# Autodesk Inventor assembly: 조립
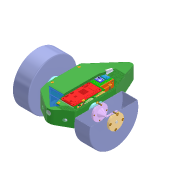
[picture p0: Inventor's stored thumbnail of the model, 180x180]
Saved by Autodesk Inventor 2020 (Build 240168000, 168)
## iProperties
Created: 2020-05-28
Part Number: 조립
Document SubType Name: Assembly
Designer: Miji
Author: Miji
## Documents named in this file (25)
- C:\Users\82102\OneDrive\바탕 화면\개인자료\졸업과제\설계\로봇\모델링 1.2\조립.iam
- C:\Users\82102\OneDrive\바탕 화면\개인자료\졸업과제\설계\로봇\모델링 1.2\본체 조립.iam
- C:\Users\82102\OneDrive\바탕 화면\개인자료\졸업과제\설계\로봇\모델링 1.2\바퀴 서브 조립.iam
- C:\Users\82102\OneDrive\바탕 화면\개인자료\졸업과제\설계\로봇\모델링 1.2\볼.ipt
- C:\Users\82102\OneDrive\바탕 화면\개인자료\졸업과제\설계\로봇\모델링 1.2\전자부품\모터.ipt
- C:\Users\82102\OneDrive\바탕 화면\개인자료\졸업과제\설계\로봇\모델링 1.2\전자부품\건전지.ipt
- C:\Users\82102\OneDrive\바탕 화면\개인자료\졸업과제\설계\로봇\모델링 1.2\전자부품\충방전\충방전.iam
- C:\Users\82102\OneDrive\바탕 화면\개인자료\졸업과제\설계\로봇\모델링 1.2\전자부품\모터드라이버\Motor Driver.ipt
- C:\Users\82102\OneDrive\바탕 화면\개인자료\졸업과제\설계\로봇\모델링 1.2\지름 핸들러.ipt
- C:\Users\82102\OneDrive\바탕 화면\개인자료\졸업과제\설계\로봇\모델링 1.2\바퀴 스퍼기어.ipt
- C:\Users\82102\OneDrive\바탕 화면\개인자료\졸업과제\설계\로봇\모델링 1.2\led 창.ipt
- C:\Users\82102\OneDrive\바탕 화면\개인자료\졸업과제\설계\로봇\모델링 1.2\카메라 창.ipt
- C:\Users\82102\OneDrive\바탕 화면\개인자료\졸업과제\설계\로봇\모델링 1.2\전자부품\카메라.ipt
- C:\Users\82102\OneDrive\바탕 화면\개인자료\졸업과제\설계\로봇\모델링 1.2\전자부품\led.ipt
- C:\Users\82102\OneDrive\바탕 화면\개인자료\졸업과제\설계\로봇\모델링 1.2\전자부품\자이로센서\MPU-9255.iam
- C:\Users\82102\OneDrive\바탕 화면\개인자료\졸업과제\설계\로봇\모델링 1.2\전자부품\아두이노 프로미니\Pro-Mini.ipt
- C:\Users\82102\OneDrive\바탕 화면\개인자료\졸업과제\설계\로봇\모델링 1.2\전자부품\로직 ic\IC CD4017.ipt
- C:\Users\82102\OneDrive\바탕 화면\개인자료\졸업과제\설계\로봇\모델링 1.2\전자부품\고도 센서\bmp180.ipt
- C:\Users\82102\OneDrive\바탕 화면\개인자료\졸업과제\설계\로봇\모델링 1.2\전자부품\raspberry-pi-zero-w\RaspberryPiZeroW.ipt
- C:\Users\82102\OneDrive\바탕 화면\개인자료\졸업과제\설계\로봇\모델링 1.2\전자부품\gps\ublox NEO-6M.iam
- C:\Users\82102\OneDrive\바탕 화면\개인자료\졸업과제\설계\로봇\모델링 1.2\전자부품\브레드 보드\20x53.ipt
- C:\Users\82102\OneDrive\바탕 화면\개인자료\졸업과제\설계\로봇\모델링 1.2\전자부품\브레드 보드\55x60.ipt
- C:\Users\82102\OneDrive\바탕 화면\개인자료\졸업과제\설계\로봇\모델링 1.2\본체 글라스.ipt
- C:\Users\82102\OneDrive\바탕 화면\개인자료\졸업과제\설계\로봇\모델링 1.2\전자부품\5v 승압 회로\Step Up.ipt
- C:\Users\82102\OneDrive\바탕 화면\개인자료\졸업과제\설계\로봇\모델링 1.2\전자부품\gps\Antenna.ipt
## Components (31 placed, 24 different names)
1. 본체 조립:1 [sub-assembly] — 메이트:1, 메이트:2, 메이트:3, 메이트:4, 메이트:5, 메이트:6, 메이트:7, 메이트:8, 메이트:9, 메이트:10, 메이트:11, 메이트:12, 메이트:13, 메이트:14, 메이트:15, 메이트:16, 메이트:17, 메이트:18, 메이트:19, 메이트:23, 메이트:24, 메이트:25, 플러쉬:1, 메이트:30, 메이트:31, 메이트:32, 메이트:33, 접선:1, 메이트:34, 각도:1, 메이트:35, 메이트:36, 플러쉬:4, 메이트:37, 메이트:38, 각도:2, 각도:3, 메이트:39, 메이트:40, 메이트:41, 메이트:42, 각도:4, 메이트:43, 각도:5, 플러쉬:5, 메이트:50, 메이트:51, 메이트:52, 각도:8, 각도:9, 메이트:58, 메이트:59, 메이트:60, 메이트:61, 메이트:62, 플러쉬:6
2. 바퀴 서브 조립:1 [sub-assembly] — 메이트:1, 메이트:2, 플러쉬:3, 회전:1
3. 바퀴 서브 조립:2 [sub-assembly] — 메이트:3, 메이트:4, 플러쉬:2, 회전:2
4. 바퀴 스퍼기어:2 — 메이트:29, 플러쉬:2, 회전:2
5. 바퀴 스퍼기어:1 — 메이트:28, 플러쉬:3, 회전:1
6. 지름 핸들러:1 — 메이트:21, 메이트:22
7. Antenna:1 — 메이트:61, 메이트:62, 플러쉬:6
8. 20x53:1 — 메이트:39, 메이트:40, 메이트:41, 메이트:53, 메이트:54, 메이트:56, 메이트:57
9. 55x60:1 — 메이트:42, 각도:4, 메이트:43, 메이트:44, 메이트:45, 메이트:46, 각도:6, 메이트:47, 메이트:48, 메이트:49, 각도:7
10. Step Up:1 — 메이트:50, 메이트:51, 메이트:52
11. MPU-9255:1 [sub-assembly] — 메이트:53, 메이트:54, 각도:8
12. Pro-Mini:1 — 메이트:46, 각도:6, 메이트:47
13. IC CD4017:1 — 메이트:48, 메이트:49, 각도:7
14. bmp180:2 — 메이트:56, 메이트:57, 각도:9
15. RaspberryPiZeroW:1 — 메이트:44, 각도:5, 메이트:45
16. ublox NEO-6M:1 [sub-assembly] — 메이트:58, 메이트:59, 메이트:60
17. led:1 — 메이트:36, 플러쉬:4, 각도:3
18. led:2 — 메이트:37, 메이트:38, 각도:2
19. 카메라:1 — 메이트:34, 각도:1, 메이트:35
20. 모터:1 — 메이트:9, 메이트:10, 메이트:11, 메이트:29
21. 모터:2 — 메이트:12, 메이트:13, 메이트:14, 메이트:21, 메이트:22
22. 모터:3 — 메이트:6, 메이트:7, 메이트:8, 메이트:28
23. 건전지:1 — 메이트:15, 메이트:16
24. 충방전:1 [sub-assembly] — 메이트:17, 메이트:18, 메이트:19
25. Motor Driver:1 — 메이트:25, 메이트:26, 메이트:27, 플러쉬:1
26. Motor Driver:2 — 메이트:23, 메이트:24, 메이트:26, 메이트:27
27. 볼:1 — 메이트:5
28. 본체 글라스:1 — 플러쉬:5
29. led 창:1 — 메이트:30
30. led 창:2 — 메이트:31, 메이트:32
31. 카메라 창:1 — 메이트:33, 접선:1
## Relationships (78: Mate 60, Angle 9, Flush 6, RelateRotation 2, Tangent 1)
- 메이트:1 [Mate]: 본체 조립:1 ↔ 바퀴 서브 조립:1
- 메이트:2 [Mate]: 본체 조립:1 ↔ 바퀴 서브 조립:1
- 메이트:3 [Mate]: 본체 조립:1 ↔ 바퀴 서브 조립:2
- 메이트:4 [Mate]: 본체 조립:1 ↔ 바퀴 서브 조립:2
- 메이트:5 [Mate]: 본체 조립:1 ↔ 볼:1
- 메이트:6 [Mate]: 본체 조립:1 ↔ 모터:3
- 메이트:7 [Mate]: 본체 조립:1 ↔ 모터:3
- 메이트:8 [Mate]: 본체 조립:1 ↔ 모터:3
- 메이트:9 [Mate]: 본체 조립:1 ↔ 모터:1
- 메이트:10 [Mate]: 본체 조립:1 ↔ 모터:1
- 메이트:11 [Mate]: 본체 조립:1 ↔ 모터:1
- 메이트:12 [Mate]: 본체 조립:1 ↔ 모터:2
- 메이트:13 [Mate]: 본체 조립:1 ↔ 모터:2
- 메이트:14 [Mate]: 본체 조립:1 ↔ 모터:2
- 메이트:15 [Mate]: 본체 조립:1 ↔ 건전지:1
- 메이트:16 [Mate]: 본체 조립:1 ↔ 건전지:1
- 메이트:17 [Mate]: 본체 조립:1 ↔ 충방전:1
- 메이트:18 [Mate]: 본체 조립:1 ↔ 충방전:1
- 메이트:19 [Mate]: 본체 조립:1 ↔ 충방전:1
- 메이트:21 [Mate]: 지름 핸들러:1 ↔ 모터:2
- 메이트:22 [Mate]: 지름 핸들러:1 ↔ 모터:2
- 메이트:23 [Mate]: 본체 조립:1 ↔ Motor Driver:2
- 메이트:24 [Mate]: 본체 조립:1 ↔ Motor Driver:2
- 메이트:25 [Mate]: 본체 조립:1 ↔ Motor Driver:1
- 메이트:26 [Mate]: Motor Driver:1 ↔ Motor Driver:2
- 메이트:27 [Mate]: Motor Driver:1 ↔ Motor Driver:2
- 플러쉬:1 [Flush] (6.5 mm): 본체 조립:1 ↔ Motor Driver:1
- 메이트:28 [Mate]: 바퀴 스퍼기어:1 ↔ 모터:3
- 메이트:29 [Mate]: 바퀴 스퍼기어:2 ↔ 모터:1
- 플러쉬:2 [Flush]: 바퀴 서브 조립:2 ↔ 바퀴 스퍼기어:2
- 플러쉬:3 [Flush]: 바퀴 서브 조립:1 ↔ 바퀴 스퍼기어:1
- 회전:1 [RelateRotation] (1 ul): 바퀴 서브 조립:1 ↔ 바퀴 스퍼기어:1
- 회전:2 [RelateRotation] (1 ul): 바퀴 서브 조립:2 ↔ 바퀴 스퍼기어:2
- 메이트:30 [Mate]: 본체 조립:1 ↔ led 창:1
- 메이트:31 [Mate]: 본체 조립:1 ↔ led 창:2
- 메이트:32 [Mate]: 본체 조립:1 ↔ led 창:2
- 메이트:33 [Mate]: 본체 조립:1 ↔ 카메라 창:1
- 접선:1 [Tangent]: 본체 조립:1 ↔ 카메라 창:1
- 메이트:34 [Mate]: 본체 조립:1 ↔ 카메라:1
- 각도:1 [Angle] (0 deg): 본체 조립:1 ↔ 카메라:1
- 메이트:35 [Mate]: 본체 조립:1 ↔ 카메라:1
- 메이트:36 [Mate]: 본체 조립:1 ↔ led:1
- 플러쉬:4 [Flush]: 본체 조립:1 ↔ led:1
- 메이트:37 [Mate]: 본체 조립:1 ↔ led:2
- 메이트:38 [Mate]: 본체 조립:1 ↔ led:2
- 각도:2 [Angle] (0 deg): 본체 조립:1 ↔ led:2
- 각도:3 [Angle] (0 deg): 본체 조립:1 ↔ led:1
- 메이트:39 [Mate]: 본체 조립:1 ↔ 20x53:1
- 메이트:40 [Mate]: 본체 조립:1 ↔ 20x53:1
- 메이트:41 [Mate]: 본체 조립:1 ↔ 20x53:1
- 메이트:42 [Mate]: 본체 조립:1 ↔ 55x60:1
- 각도:4 [Angle] (0 deg): 본체 조립:1 ↔ 55x60:1
- 메이트:43 [Mate]: 본체 조립:1 ↔ 55x60:1
- 메이트:44 [Mate]: 55x60:1 ↔ RaspberryPiZeroW:1
- 각도:5 [Angle] (0 deg): 본체 조립:1 ↔ RaspberryPiZeroW:1
- 메이트:45 [Mate]: 55x60:1 ↔ RaspberryPiZeroW:1
- 플러쉬:5 [Flush]: 본체 조립:1 ↔ 본체 글라스:1
- 메이트:46 [Mate]: 55x60:1 ↔ Pro-Mini:1
- 각도:6 [Angle] (0 deg): 55x60:1 ↔ Pro-Mini:1
- 메이트:47 [Mate]: 55x60:1 ↔ Pro-Mini:1
- 메이트:48 [Mate]: 55x60:1 ↔ IC CD4017:1
- 메이트:49 [Mate]: 55x60:1 ↔ IC CD4017:1
- 각도:7 [Angle] (0 deg): 55x60:1 ↔ IC CD4017:1
- 메이트:50 [Mate]: 본체 조립:1 ↔ Step Up:1
- 메이트:51 [Mate]: 본체 조립:1 ↔ Step Up:1
- 메이트:52 [Mate]: 본체 조립:1 ↔ Step Up:1
- 메이트:53 [Mate]: 20x53:1 ↔ MPU-9255:1
- 메이트:54 [Mate]: 20x53:1 ↔ MPU-9255:1
- 각도:8 [Angle] (0 deg): 본체 조립:1 ↔ MPU-9255:1
- 메이트:56 [Mate]: 20x53:1 ↔ bmp180:2
- 메이트:57 [Mate]: 20x53:1 ↔ bmp180:2
- 각도:9 [Angle] (0 deg): 본체 조립:1 ↔ bmp180:2
- 메이트:58 [Mate]: 본체 조립:1 ↔ ublox NEO-6M:1
- 메이트:59 [Mate]: 본체 조립:1 ↔ ublox NEO-6M:1
- 메이트:60 [Mate]: 본체 조립:1 ↔ ublox NEO-6M:1
- 메이트:61 [Mate]: 본체 조립:1 ↔ Antenna:1
- 메이트:62 [Mate]: 본체 조립:1 ↔ Antenna:1
- 플러쉬:6 [Flush] (-1 mm): 본체 조립:1 ↔ Antenna:1
